# Autodesk Inventor assembly: final ss
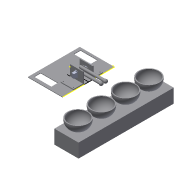
[picture p0: Inventor's stored thumbnail of the model, 180x180]
Saved by Autodesk Inventor 2019 (Build 230136000, 136)
## iProperties
Created: 2020-03-06
Part Number: final ss
Document SubType Name: Assembly
Designer: Pranav naik
Author: Pranav naik
## Documents named in this file (12)
- C:\Users\Pranan A Naik\Documents\final ss.iam
- C:\Users\Pranan A Naik\Documents\pice.ipt
- C:\Users\Pranan A Naik\Documents\stik.ipt
- C:\Users\Pranan A Naik\Documents\clamp2.ipt
- C:\Users\Pranan A Naik\Documents\servomotor.ipt
- C:\Users\Pranan A Naik\Documents\base.ipt
- C:\Users\Pranan A Naik\Documents\clamp2_MIR.ipt
- C:\Users\Pranan A Naik\Documents\servomotor_MIR1.ipt
- C:\Users\Pranan A Naik\Documents\pice_MIR1.ipt
- C:\Users\Pranan A Naik\Documents\stik_MIR1.ipt
- C:\Users\Pranan A Naik\Documents\stand.ipt
- C:\Users\Pranan A Naik\Documents\bowl.ipt
## Components (14 placed, 11 different names)
1. clamp2:1
2. servomotor:3 — Insert:1
3. pice:1 — Insert:1
4. stik:1
5. base:1
6. clamp2_MIR:1
7. servomotor_MIR1:1 — Insert:2
8. pice_MIR1:1 — Insert:2
9. stik_MIR1:1
10. stand:1
11. bowl:1
12. bowl:2
13. bowl:3
14. bowl:4
## Relationships (2: Insert 2)
- Insert:1: servomotor:3 ↔ pice:1
- Insert:2: servomotor_MIR1:1 ↔ pice_MIR1:1
